# Autodesk Inventor assembly: IndexerPolyWheelPlateSet_MIR
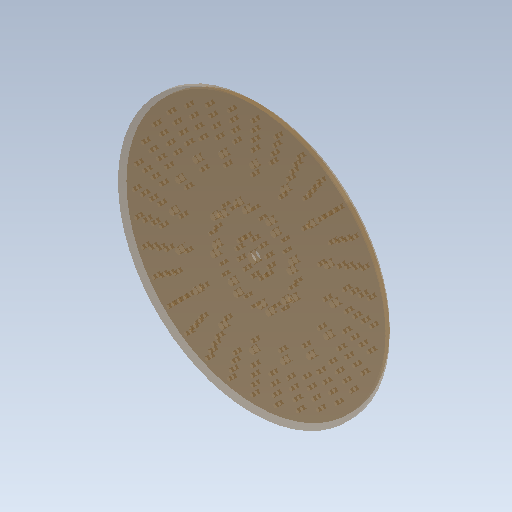
[picture p0: Inventor's stored thumbnail of the model, 512x512]
Saved by Autodesk Inventor 2020 (Build 240168000, 168)
## iProperties
Created: 2020-01-19
Part Number: IndexerPolyWheelPlateSet_MIR
Document SubType Name: Assembly
Designer: srini
Author: srini
## Documents named in this file (3)
- C:\Users\srini\Documents\FRC\2020\IntakeShooter\IndexerPolyWheelPlateSet_MIR.iam
- C:\Users\srini\Documents\FRC\2020\IntakeShooter\IndexWheelFlatPlatesPolyOutside_MIR.ipt
- C:\Users\srini\Documents\FRC\2020\IntakeShooter\IndexWheelFlatPlatesPolyInside_MIR.ipt
## Components (2 placed, 2 different names)
1. IndexWheelFlatPlatesPolyOutside_MIR:1 — Insert:2, Insert:1
2. IndexWheelFlatPlatesPolyInside_MIR:1 — Insert:2, Insert:1
## Relationships (2: Insert 2)
- Insert:2: IndexWheelFlatPlatesPolyOutside_MIR:1 ↔ IndexWheelFlatPlatesPolyInside_MIR:1
- Insert:1: IndexWheelFlatPlatesPolyOutside_MIR:1 ↔ IndexWheelFlatPlatesPolyInside_MIR:1
